# Autodesk Inventor assembly: Field Crater Side left mineral FACING WRONG WAY
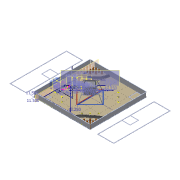
[picture p0: Inventor's stored thumbnail of the model, 180x180]
Saved by Autodesk Inventor 2018 (Build 220112000, 112)
## iProperties
Created: 2018-08-21
Part Number: Field Crater Side left mineral FACING WRONG WAY
Description: STEP AP214
Document SubType Name: Assembly
Designer: ball
Sending System: SolidWorks 2018
Preprocessor: SwSTEP 2.0
Title: Production Full Field 0-2 Final Final.STEP
Revision Number: ANY
## Documents named in this file (13)
- C:\FTC\FTC8863CAD\2018Robot\Field\Field Crater Side left mineral FACING WRONG WAY.iam
- C:\FTC\FTC8863CAD\2018Robot\Field\Perimeter and Tiles.iam
- C:\FTC\FTC8863CAD\2018Robot\Field\Corner Crater Rim.iam
- C:\FTC\FTC8863CAD\2018Robot\Field\Player Station.ipt
- C:\FTC\FTC8863CAD\2018Robot\Field\Production Lander.iam
- C:\FTC\FTC8863CAD\2018Robot\Field\Center Diamond.ipt
- C:\FTC\FTC8863CAD\2018Robot\Field\1 tile safe zone.ipt
- C:\FTC\FTC8863CAD\2018Robot\Field\Sample Field.ipt
- C:\FTC\FTC8863CAD\2018Robot\Field\Game Piece Array.iam
- C:\FTC\FTC8863CAD\2018Robot\Field\Target in sleeve.ipt
- C:\FTC\FTC8863CAD\2018Robot\Field\robot.ipt
- C:\FTC\FTC8863CAD\2018Robot\Field\am-2850 wiffle base Ball.ipt
- C:\FTC\FTC8863CAD\2018Robot\Field\Lanes.ipt
## Components (31 placed, 24 different names)
1. Perimeter and Tiles_1 [sub-assembly] — Mate:1, Flush:2, Mate:7, Mate:9, Mate:11, Flush:4, Mate:14, Mate:20, Mate:22
2. Corner Crater Rim_2 [sub-assembly]
3. Corner Crater Rim_3 [sub-assembly]
4. Player Station_4
5. Player Station_5
6. Production Lander_6 [sub-assembly] — Angle:1, Mate:2, Flush:3, Mate:13
7. Center Diamond_7
8. 1 tile safe zone_8
9. 1 tile safe zone_9
10. Sample Field_10 — Mate:5
11. Sample Field_11
12. Sample Field_12
13. Sample Field_13
14. 1 tile safe zone_14
15. 1 tile safe zone_15
16. Game Piece Array_16 [sub-assembly]
17. Game Piece Array_17 [sub-assembly]
18. Target in sleeve_18
19. Target in sleeve_19
20. Target in sleeve_20
21. Target in sleeve_21
22. robot:1 — Mate:1, Angle:1, Mate:2, Mate:13, Angle:2, Mate:17
23. am-2850 wiffle base Ball:1 — Mate:5
24. am-2850 wiffle base Ball:2
25. Lanes:1 — Flush:2
26. robot:3 — Mate:7, Mate:18, Mate:19, Mate:21
27. robot:4 — Mate:9
28. robot:5 — Mate:11, Angle:2, Mate:16, Mate:17, Mate:18, Mate:19
29. robot:6 — Mate:14, Mate:15
30. robot:7 — Mate:20, Mate:21, Mate:24
31. robot:8 — Mate:22, Mate:23, Mate:24
## Relationships (23: Mate 18, Flush 3, Angle 2)
- Mate:1: Perimeter and Tiles_1 ↔ robot:1
- Angle:1 (0 deg): Production Lander_6 ↔ robot:1
- Mate:2 (15.24 mm): Production Lander_6 ↔ robot:1
- Mate:5: Sample Field_10 ↔ am-2850 wiffle base Ball:1
- Flush:2: Perimeter and Tiles_1 ↔ Lanes:1
- Mate:7: Perimeter and Tiles_1 ↔ robot:3
- Mate:9: Perimeter and Tiles_1 ↔ robot:4
- Mate:11: Perimeter and Tiles_1 ↔ robot:5
- Flush:3 (611.3272 mm): Production Lander_6
- Flush:4 (293.0652 mm): Perimeter and Tiles_1
- Mate:13 (-53.975 mm): Production Lander_6 ↔ robot:1
- Mate:14: Perimeter and Tiles_1 ↔ robot:6
- Mate:15: robot:6
- Angle:2 (90 deg): robot:1 ↔ robot:5
- Mate:16 (-153.67 mm): robot:5
- Mate:17 (-214.3506 mm): robot:1 ↔ robot:5
- Mate:18 (214.3506 mm): robot:3 ↔ robot:5
- Mate:19 (-214.3506 mm): robot:3 ↔ robot:5
- Mate:20: Perimeter and Tiles_1 ↔ robot:7
- Mate:21: robot:3 ↔ robot:7
- Mate:22: Perimeter and Tiles_1 ↔ robot:8
- Mate:23: robot:8
- Mate:24 (215.392 mm): robot:7 ↔ robot:8
